# Autodesk Inventor assembly: Alternate Z belt Sub
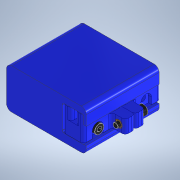
[picture p0: Inventor's stored thumbnail of the model, 180x180]
Saved by Autodesk Inventor 2022 (Build 260153000, 153)
## iProperties
Created: 2022-03-26
Part Number: Alternate Z belt Sub
Document SubType Name: Assembly
Designer: Nick
Author: Nick
## Documents named in this file (6)
- Y:\Projects\Bibble0\SubAsm\Alternate Z belt Sub.iam
- Y:\Projects\Bibble0\3D printed\Z Axis\Z Belt Tensioner HSI.iam
- Y:\Projects\Bibble0\Hardware\M3 x 14 mm  SHCS.ipt
- Y:\Projects\Bibble0\3D printed\Z Axis\Z Belt Tensioner - Mirror HSI.iam
- Y:\Projects\Bibble0\Hardware\M3 x 10 mm FHCS.ipt
- Y:\Projects\Bibble0\3D printed\Z Axis\Alternate Z Belt Housing HSI.iam
## Components (7 placed, 5 different names)
1. Z Belt Tensioner HSI:1 [sub-assembly]
2. Alternate Z Belt Housing HSI:1 [sub-assembly] — Angle:1
3. M3 x 14 mm  SHCS:1
4. Z Belt Tensioner - Mirror HSI:1 [sub-assembly] — Angle:1
5. M3 x 10 mm FHCS:1
6. M3 x 10 mm FHCS:2
7. M3 x 14 mm  SHCS:2
## Relationships (10: Insert 4, Flush 3, Mate 2, Angle 1)
- [Insert] (0.2 mm): Z Belt Tensioner HSI:1 ↔ Alternate Z Belt Housing HSI:1
- [Insert]: Z Belt Tensioner HSI:1 ↔ M3 x 14 mm  SHCS:1
- [Insert]: Z Belt Tensioner HSI:1 ↔ Z Belt Tensioner - Mirror HSI:1
- [Flush]: Z Belt Tensioner HSI:1 ↔ Z Belt Tensioner - Mirror HSI:1
- [Flush]: Z Belt Tensioner HSI:1 ↔ M3 x 10 mm FHCS:1
- [Flush]: Z Belt Tensioner - Mirror HSI:1 ↔ M3 x 10 mm FHCS:2
- [Mate]: Z Belt Tensioner - Mirror HSI:1 ↔ M3 x 10 mm FHCS:2
- [Mate]: Z Belt Tensioner HSI:1 ↔ M3 x 10 mm FHCS:1
- [Insert]: Z Belt Tensioner - Mirror HSI:1 ↔ M3 x 14 mm  SHCS:2
- Angle:1 (0 deg): Alternate Z Belt Housing HSI:1 ↔ Z Belt Tensioner - Mirror HSI:1
